# Autodesk Inventor assembly: poleAssembly
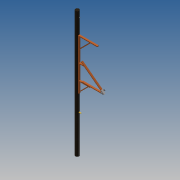
[picture p0: Inventor's stored thumbnail of the model, 180x180]
Saved by Autodesk Inventor 2014 SP1 (Build 180222100, 222)
## iProperties
Created: 2014-08-25
Part Number: poleAssembly
Document SubType Name: Assembly
Designer: Dave
Author: Dave
## Documents named in this file (6)
- C:\Users\Dave\Desktop\hera-cad\Node\poleAssembly.iam
- C:\Users\Dave\Desktop\hera-cad\support\pole.ipt
- C:\Users\Dave\Desktop\hera-cad\support\heightMarker.ipt
- C:\Users\Dave\Desktop\hera-cad\support\poleStandVertAssy.iam
- C:\Users\Dave\Desktop\hera-cad\support\poleStandHorizAssy.iam
- C:\Users\Dave\Desktop\hera-cad\smallParts\eyebolt_ss_375.ipt
## Components (5 placed, 5 different names)
1. pole:1 — Insert:1, Mate:4, Flush:2, Insert:2
2. heightMarker:1 — Insert:1, Mate:1
3. poleStandVertAssy:1 [sub-assembly] — Mate:1, Mate:2, Flush:1, Mate:3, Mate:4, Flush:2
4. poleStandHorizAssy:1 [sub-assembly] — Mate:2, Flush:1, Mate:3
5. eyebolt_ss_375:1 — Insert:2
## Relationships (8: Mate 4, Insert 2, Flush 2)
- Insert:1 (-2143.76 mm): pole:1 ↔ heightMarker:1
- Mate:1 (908.05 mm): heightMarker:1 ↔ poleStandVertAssy:1
- Mate:2: poleStandVertAssy:1 ↔ poleStandHorizAssy:1
- Flush:1: poleStandVertAssy:1 ↔ poleStandHorizAssy:1
- Mate:3 (150.6728 mm): poleStandVertAssy:1 ↔ poleStandHorizAssy:1
- Mate:4: pole:1 ↔ poleStandVertAssy:1
- Flush:2 (60.96 mm): pole:1 ↔ poleStandVertAssy:1
- Insert:2 (-50.8 mm): pole:1 ↔ eyebolt_ss_375:1
